# Autodesk Inventor assembly: Deposito
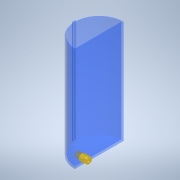
[picture p0: Inventor's stored thumbnail of the model, 180x180]
Saved by Autodesk Inventor 2020 (Build 240168000, 168)
## iProperties
Created: 2020-10-28
Part Number: Deposito
Document SubType Name: Assembly
Designer: aaron
Author: aaron
## Documents named in this file (3)
- C:\Users\aaron\OneDrive\Escritorio\Proyecto\Deposito.iam
- C:\Users\aaron\OneDrive\Escritorio\Proyecto\Deposito_Líquido.ipt
- C:\Users\aaron\OneDrive\Escritorio\Proyecto\ConectorPTFE_4.ipt
## Components (2 placed, 2 different names)
1. Deposito_Líquido:1 — Mate:1, Mate:2
2. ConectorPTFE_4:1 — Mate:1, Mate:2
## Relationships (2: Mate 2)
- Mate:1: Deposito_Líquido:1 ↔ ConectorPTFE_4:1
- Mate:2: Deposito_Líquido:1 ↔ ConectorPTFE_4:1
